# Autodesk Inventor assembly: FrontMountAssembly_SimplifiedVersion
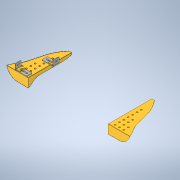
[picture p0: Inventor's stored thumbnail of the model, 180x180]
Saved by Autodesk Inventor 2021 (Build 250183000, 183)
## iProperties
Created: 2019-05-05
Part Number: FrontMountAssembly_SimplifiedVersion
Document SubType Name: Assembly
Designer: lgnds
Author: lgnds
## Documents named in this file (3)
- C:\Users\Viktor\Google Drive\Chalmers\Fortsatt arbete WR\Design files\FRS - Front Rail System_V2\FästenFörRam\FrontMountAssembly_SimplifiedVersion.iam
- C:\Users\Viktor\Google Drive\Chalmers\Fortsatt arbete WR\Design files\FRS - Front Rail System_V2\FästenFörRam\FrontMountVersion2_SimplifiedVersion.ipt
- C:\Users\Viktor\Google Drive\Chalmers\Fortsatt arbete WR\Design files\FRS - Front Rail System_V2\FästenFörRam\FrontMountVersion2_SimplifiedVersion_MIR.ipt
## Components (2 placed, 2 different names)
1. FrontMountVersion2_SimplifiedVersion:1 — Mate:1, Mate:2, Flush:1
2. FrontMountVersion2_SimplifiedVersion_MIR:1 — Flush:5, Mate:12, Flush:6
## Relationships (6: Mate 3, Flush 3)
- Mate:1 (183 mm): FrontMountVersion2_SimplifiedVersion:1
- Mate:2: FrontMountVersion2_SimplifiedVersion:1
- Flush:1 (-45 mm): FrontMountVersion2_SimplifiedVersion:1
- Flush:5 (-45 mm): FrontMountVersion2_SimplifiedVersion_MIR:1
- Mate:12: FrontMountVersion2_SimplifiedVersion_MIR:1
- Flush:6 (-183 mm): FrontMountVersion2_SimplifiedVersion_MIR:1
